# Autodesk Inventor assembly: Assembly
(part 2 of 3)
- C:\Users\Vincent Larson\Downloads\Universal_board_70x90mm_31x26\Universal_board_70x90mm_31x26-prt461.ipt
- C:\Users\Vincent Larson\Downloads\Universal_board_70x90mm_31x26\Universal_board_70x90mm_31x26-prt462.ipt
- C:\Users\Vincent Larson\Downloads\Universal_board_70x90mm_31x26\Universal_board_70x90mm_31x26-prt463.ipt
- C:\Users\Vincent Larson\Downloads\Universal_board_70x90mm_31x26\Universal_board_70x90mm_31x26-prt464.ipt
- C:\Users\Vincent Larson\Downloads\Universal_board_70x90mm_31x26\Universal_board_70x90mm_31x26-prt465.ipt
- C:\Users\Vincent Larson\Downloads\Universal_board_70x90mm_31x26\Universal_board_70x90mm_31x26-prt466.ipt
- C:\Users\Vincent Larson\Downloads\Universal_board_70x90mm_31x26\Universal_board_70x90mm_31x26-prt467.ipt
- C:\Users\Vincent Larson\Downloads\Universal_board_70x90mm_31x26\Universal_board_70x90mm_31x26-prt468.ipt
- C:\Users\Vincent Larson\Downloads\Universal_board_70x90mm_31x26\Universal_board_70x90mm_31x26-prt469.ipt
- C:\Users\Vincent Larson\Downloads\Universal_board_70x90mm_31x26\Universal_board_70x90mm_31x26-prt470.ipt
- C:\Users\Vincent Larson\Downloads\Universal_board_70x90mm_31x26\Universal_board_70x90mm_31x26-prt471.ipt
- C:\Users\Vincent Larson\Downloads\Universal_board_70x90mm_31x26\Universal_board_70x90mm_31x26-prt472.ipt
- C:\Users\Vincent Larson\Downloads\Universal_board_70x90mm_31x26\Universal_board_70x90mm_31x26-prt473.ipt
- C:\Users\Vincent Larson\Downloads\Universal_board_70x90mm_31x26\Universal_board_70x90mm_31x26-prt474.ipt
- C:\Users\Vincent Larson\Downloads\Universal_board_70x90mm_31x26\Universal_board_70x90mm_31x26-prt475.ipt
- C:\Users\Vincent Larson\Downloads\Universal_board_70x90mm_31x26\Universal_board_70x90mm_31x26-prt476.ipt
- C:\Users\Vincent Larson\Downloads\Universal_board_70x90mm_31x26\Universal_board_70x90mm_31x26-prt477.ipt
- C:\Users\Vincent Larson\Downloads\Universal_board_70x90mm_31x26\Universal_board_70x90mm_31x26-prt478.ipt
- C:\Users\Vincent Larson\Downloads\Universal_board_70x90mm_31x26\Universal_board_70x90mm_31x26-prt479.ipt
- C:\Users\Vincent Larson\Downloads\Universal_board_70x90mm_31x26\Universal_board_70x90mm_31x26-prt480.ipt
- C:\Users\Vincent Larson\Downloads\Universal_board_70x90mm_31x26\Universal_board_70x90mm_31x26-prt481.ipt
- C:\Users\Vincent Larson\Downloads\Universal_board_70x90mm_31x26\Universal_board_70x90mm_31x26-prt482.ipt
- C:\Users\Vincent Larson\Downloads\Universal_board_70x90mm_31x26\Universal_board_70x90mm_31x26-prt483.ipt
- C:\Users\Vincent Larson\Downloads\Universal_board_70x90mm_31x26\Universal_board_70x90mm_31x26-prt484.ipt
- C:\Users\Vincent Larson\Downloads\Universal_board_70x90mm_31x26\Universal_board_70x90mm_31x26-prt485.ipt
- C:\Users\Vincent Larson\Downloads\Universal_board_70x90mm_31x26\Universal_board_70x90mm_31x26-prt486.ipt
- C:\Users\Vincent Larson\Downloads\Universal_board_70x90mm_31x26\Universal_board_70x90mm_31x26-prt487.ipt
- C:\Users\Vincent Larson\Downloads\Universal_board_70x90mm_31x26\Universal_board_70x90mm_31x26-prt488.ipt
- C:\Users\Vincent Larson\Downloads\Universal_board_70x90mm_31x26\Universal_board_70x90mm_31x26-prt489.ipt
- C:\Users\Vincent Larson\Downloads\Universal_board_70x90mm_31x26\Universal_board_70x90mm_31x26-prt490.ipt
- C:\Users\Vincent Larson\Downloads\Universal_board_70x90mm_31x26\Universal_board_70x90mm_31x26-prt491.ipt
- C:\Users\Vincent Larson\Downloads\Universal_board_70x90mm_31x26\Universal_board_70x90mm_31x26-prt492.ipt
- C:\Users\Vincent Larson\Downloads\Universal_board_70x90mm_31x26\Universal_board_70x90mm_31x26-prt493.ipt
- C:\Users\Vincent Larson\Downloads\Universal_board_70x90mm_31x26\Universal_board_70x90mm_31x26-prt494.ipt
- C:\Users\Vincent Larson\Downloads\Universal_board_70x90mm_31x26\Universal_board_70x90mm_31x26-prt495.ipt
- C:\Users\Vincent Larson\Downloads\Universal_board_70x90mm_31x26\Universal_board_70x90mm_31x26-prt496.ipt
- C:\Users\Vincent Larson\Downloads\Universal_board_70x90mm_31x26\Universal_board_70x90mm_31x26-prt497.ipt
- C:\Users\Vincent Larson\Downloads\Universal_board_70x90mm_31x26\Universal_board_70x90mm_31x26-prt498.ipt
- C:\Users\Vincent Larson\Downloads\Universal_board_70x90mm_31x26\Universal_board_70x90mm_31x26-prt499.ipt
- C:\Users\Vincent Larson\Downloads\Universal_board_70x90mm_31x26\Universal_board_70x90mm_31x26-prt500.ipt
- C:\Users\Vincent Larson\Downloads\Universal_board_70x90mm_31x26\Universal_board_70x90mm_31x26-prt501.ipt
- C:\Users\Vincent Larson\Downloads\Universal_board_70x90mm_31x26\Universal_board_70x90mm_31x26-prt502.ipt
- C:\Users\Vincent Larson\Downloads\Universal_board_70x90mm_31x26\Universal_board_70x90mm_31x26-prt503.ipt
- C:\Users\Vincent Larson\Downloads\Universal_board_70x90mm_31x26\Universal_board_70x90mm_31x26-prt504.ipt
- C:\Users\Vincent Larson\Downloads\Universal_board_70x90mm_31x26\Universal_board_70x90mm_31x26-prt505.ipt
- C:\Users\Vincent Larson\Downloads\Universal_board_70x90mm_31x26\Universal_board_70x90mm_31x26-prt506.ipt
- C:\Users\Vincent Larson\Downloads\Universal_board_70x90mm_31x26\Universal_board_70x90mm_31x26-prt507.ipt
- C:\Users\Vincent Larson\Downloads\Universal_board_70x90mm_31x26\Universal_board_70x90mm_31x26-prt508.ipt
- C:\Users\Vincent Larson\Downloads\Universal_board_70x90mm_31x26\Universal_board_70x90mm_31x26-prt509.ipt
- C:\Users\Vincent Larson\Downloads\Universal_board_70x90mm_31x26\Universal_board_70x90mm_31x26-prt510.ipt
- C:\Users\Vincent Larson\Downloads\Universal_board_70x90mm_31x26\Universal_board_70x90mm_31x26-prt511.ipt
- C:\Users\Vincent Larson\Downloads\Universal_board_70x90mm_31x26\Universal_board_70x90mm_31x26-prt512.ipt
- C:\Users\Vincent Larson\Downloads\Universal_board_70x90mm_31x26\Universal_board_70x90mm_31x26-prt513.ipt
- C:\Users\Vincent Larson\Downloads\Universal_board_70x90mm_31x26\Universal_board_70x90mm_31x26-prt514.ipt
- C:\Users\Vincent Larson\Downloads\Universal_board_70x90mm_31x26\Universal_board_70x90mm_31x26-prt515.ipt
- C:\Users\Vincent Larson\Downloads\Universal_board_70x90mm_31x26\Universal_board_70x90mm_31x26-prt516.ipt
- C:\Users\Vincent Larson\Downloads\Universal_board_70x90mm_31x26\Universal_board_70x90mm_31x26-prt517.ipt
- C:\Users\Vincent Larson\Downloads\Universal_board_70x90mm_31x26\Universal_board_70x90mm_31x26-prt518.ipt
- C:\Users\Vincent Larson\Downloads\Universal_board_70x90mm_31x26\Universal_board_70x90mm_31x26-prt519.ipt
- C:\Users\Vincent Larson\Downloads\Universal_board_70x90mm_31x26\Universal_board_70x90mm_31x26-prt520.ipt
- C:\Users\Vincent Larson\Downloads\Universal_board_70x90mm_31x26\Universal_board_70x90mm_31x26-prt521.ipt
- C:\Users\Vincent Larson\Downloads\Universal_board_70x90mm_31x26\Universal_board_70x90mm_31x26-prt522.ipt
- C:\Users\Vincent Larson\Downloads\Universal_board_70x90mm_31x26\Universal_board_70x90mm_31x26-prt523.ipt
- C:\Users\Vincent Larson\Downloads\Universal_board_70x90mm_31x26\Universal_board_70x90mm_31x26-prt524.ipt
- C:\Users\Vincent Larson\Downloads\Universal_board_70x90mm_31x26\Universal_board_70x90mm_31x26-prt525.ipt
- C:\Users\Vincent Larson\Downloads\Universal_board_70x90mm_31x26\Universal_board_70x90mm_31x26-prt526.ipt
- C:\Users\Vincent Larson\Downloads\Universal_board_70x90mm_31x26\Universal_board_70x90mm_31x26-prt527.ipt
- C:\Users\Vincent Larson\Downloads\Universal_board_70x90mm_31x26\Universal_board_70x90mm_31x26-prt528.ipt
- C:\Users\Vincent Larson\Downloads\Universal_board_70x90mm_31x26\Universal_board_70x90mm_31x26-prt529.ipt
- C:\Users\Vincent Larson\Downloads\Universal_board_70x90mm_31x26\Universal_board_70x90mm_31x26-prt530.ipt
- C:\Users\Vincent Larson\Downloads\Universal_board_70x90mm_31x26\Universal_board_70x90mm_31x26-prt531.ipt
- C:\Users\Vincent Larson\Downloads\Universal_board_70x90mm_31x26\Universal_board_70x90mm_31x26-prt532.ipt
- C:\Users\Vincent Larson\Downloads\Universal_board_70x90mm_31x26\Universal_board_70x90mm_31x26-prt533.ipt
- C:\Users\Vincent Larson\Downloads\Universal_board_70x90mm_31x26\Universal_board_70x90mm_31x26-prt534.ipt
- C:\Users\Vincent Larson\Downloads\Universal_board_70x90mm_31x26\Universal_board_70x90mm_31x26-prt535.ipt
- C:\Users\Vincent Larson\Downloads\Universal_board_70x90mm_31x26\Universal_board_70x90mm_31x26-prt536.ipt
- C:\Users\Vincent Larson\Downloads\Universal_board_70x90mm_31x26\Universal_board_70x90mm_31x26-prt537.ipt
- C:\Users\Vincent Larson\Downloads\Universal_board_70x90mm_31x26\Universal_board_70x90mm_31x26-prt538.ipt
- C:\Users\Vincent Larson\Downloads\Universal_board_70x90mm_31x26\Universal_board_70x90mm_31x26-prt539.ipt
- C:\Users\Vincent Larson\Downloads\Universal_board_70x90mm_31x26\Universal_board_70x90mm_31x26-prt540.ipt
- C:\Users\Vincent Larson\Downloads\Universal_board_70x90mm_31x26\Universal_board_70x90mm_31x26-prt541.ipt
- C:\Users\Vincent Larson\Downloads\Universal_board_70x90mm_31x26\Universal_board_70x90mm_31x26-prt542.ipt
- C:\Users\Vincent Larson\Downloads\Universal_board_70x90mm_31x26\Universal_board_70x90mm_31x26-prt543.ipt
- C:\Users\Vincent Larson\Downloads\Universal_board_70x90mm_31x26\Universal_board_70x90mm_31x26-prt544.ipt
- C:\Users\Vincent Larson\Downloads\Universal_board_70x90mm_31x26\Universal_board_70x90mm_31x26-prt545.ipt
- C:\Users\Vincent Larson\Downloads\Universal_board_70x90mm_31x26\Universal_board_70x90mm_31x26-prt546.ipt
- C:\Users\Vincent Larson\Downloads\Universal_board_70x90mm_31x26\Universal_board_70x90mm_31x26-prt547.ipt
- C:\Users\Vincent Larson\Downloads\Universal_board_70x90mm_31x26\Universal_board_70x90mm_31x26-prt548.ipt
- C:\Users\Vincent Larson\Downloads\Universal_board_70x90mm_31x26\Universal_board_70x90mm_31x26-prt549.ipt
- C:\Users\Vincent Larson\Downloads\Universal_board_70x90mm_31x26\Universal_board_70x90mm_31x26-prt550.ipt
- C:\Users\Vincent Larson\Downloads\Universal_board_70x90mm_31x26\Universal_board_70x90mm_31x26-prt551.ipt
- C:\Users\Vincent Larson\Downloads\Universal_board_70x90mm_31x26\Universal_board_70x90mm_31x26-prt552.ipt
- C:\Users\Vincent Larson\Downloads\Universal_board_70x90mm_31x26\Universal_board_70x90mm_31x26-prt553.ipt
- C:\Users\Vincent Larson\Downloads\Universal_board_70x90mm_31x26\Universal_board_70x90mm_31x26-prt554.ipt
- C:\Users\Vincent Larson\Downloads\Universal_board_70x90mm_31x26\Universal_board_70x90mm_31x26-prt555.ipt
- C:\Users\Vincent Larson\Downloads\Universal_board_70x90mm_31x26\Universal_board_70x90mm_31x26-prt556.ipt
- C:\Users\Vincent Larson\Downloads\Universal_board_70x90mm_31x26\Universal_board_70x90mm_31x26-prt557.ipt
- C:\Users\Vincent Larson\Downloads\Universal_board_70x90mm_31x26\Universal_board_70x90mm_31x26-prt558.ipt
- C:\Users\Vincent Larson\Downloads\Universal_board_70x90mm_31x26\Universal_board_70x90mm_31x26-prt559.ipt
- C:\Users\Vincent Larson\Downloads\Universal_board_70x90mm_31x26\Universal_board_70x90mm_31x26-prt560.ipt
- C:\Users\Vincent Larson\Downloads\Universal_board_70x90mm_31x26\Universal_board_70x90mm_31x26-prt561.ipt
- C:\Users\Vincent Larson\Downloads\Universal_board_70x90mm_31x26\Universal_board_70x90mm_31x26-prt562.ipt
- C:\Users\Vincent Larson\Downloads\Universal_board_70x90mm_31x26\Universal_board_70x90mm_31x26-prt563.ipt
- C:\Users\Vincent Larson\Downloads\Universal_board_70x90mm_31x26\Universal_board_70x90mm_31x26-prt564.ipt
- C:\Users\Vincent Larson\Downloads\Universal_board_70x90mm_31x26\Universal_board_70x90mm_31x26-prt565.ipt
- C:\Users\Vincent Larson\Downloads\Universal_board_70x90mm_31x26\Universal_board_70x90mm_31x26-prt566.ipt
- C:\Users\Vincent Larson\Downloads\Universal_board_70x90mm_31x26\Universal_board_70x90mm_31x26-prt567.ipt
- C:\Users\Vincent Larson\Downloads\Universal_board_70x90mm_31x26\Universal_board_70x90mm_31x26-prt568.ipt
- C:\Users\Vincent Larson\Downloads\Universal_board_70x90mm_31x26\Universal_board_70x90mm_31x26-prt569.ipt
- C:\Users\Vincent Larson\Downloads\Universal_board_70x90mm_31x26\Universal_board_70x90mm_31x26-prt570.ipt
- C:\Users\Vincent Larson\Downloads\Universal_board_70x90mm_31x26\Universal_board_70x90mm_31x26-prt571.ipt
- C:\Users\Vincent Larson\Downloads\Universal_board_70x90mm_31x26\Universal_board_70x90mm_31x26-prt572.ipt
- C:\Users\Vincent Larson\Downloads\Universal_board_70x90mm_31x26\Universal_board_70x90mm_31x26-prt573.ipt
- C:\Users\Vincent Larson\Downloads\Universal_board_70x90mm_31x26\Universal_board_70x90mm_31x26-prt574.ipt
- C:\Users\Vincent Larson\Downloads\Universal_board_70x90mm_31x26\Universal_board_70x90mm_31x26-prt575.ipt
- C:\Users\Vincent Larson\Downloads\Universal_board_70x90mm_31x26\Universal_board_70x90mm_31x26-prt576.ipt
- C:\Users\Vincent Larson\Downloads\Universal_board_70x90mm_31x26\Universal_board_70x90mm_31x26-prt577.ipt
- C:\Users\Vincent Larson\Downloads\Universal_board_70x90mm_31x26\Universal_board_70x90mm_31x26-prt578.ipt
- C:\Users\Vincent Larson\Downloads\Universal_board_70x90mm_31x26\Universal_board_70x90mm_31x26-prt579.ipt
- C:\Users\Vincent Larson\Downloads\Universal_board_70x90mm_31x26\Universal_board_70x90mm_31x26-prt580.ipt
- C:\Users\Vincent Larson\Downloads\Universal_board_70x90mm_31x26\Universal_board_70x90mm_31x26-prt581.ipt
- C:\Users\Vincent Larson\Downloads\Universal_board_70x90mm_31x26\Universal_board_70x90mm_31x26-prt582.ipt
- C:\Users\Vincent Larson\Downloads\Universal_board_70x90mm_31x26\Universal_board_70x90mm_31x26-prt583.ipt
- C:\Users\Vincent Larson\Downloads\Universal_board_70x90mm_31x26\Universal_board_70x90mm_31x26-prt584.ipt
- C:\Users\Vincent Larson\Downloads\Universal_board_70x90mm_31x26\Universal_board_70x90mm_31x26-prt585.ipt
- C:\Users\Vincent Larson\Downloads\Universal_board_70x90mm_31x26\Universal_board_70x90mm_31x26-prt586.ipt
- C:\Users\Vincent Larson\Downloads\Universal_board_70x90mm_31x26\Universal_board_70x90mm_31x26-prt587.ipt
- C:\Users\Vincent Larson\Downloads\Universal_board_70x90mm_31x26\Universal_board_70x90mm_31x26-prt588.ipt
- C:\Users\Vincent Larson\Downloads\Universal_board_70x90mm_31x26\Universal_board_70x90mm_31x26-prt589.ipt
- C:\Users\Vincent Larson\Downloads\Universal_board_70x90mm_31x26\Universal_board_70x90mm_31x26-prt590.ipt
- C:\Users\Vincent Larson\Downloads\Universal_board_70x90mm_31x26\Universal_board_70x90mm_31x26-prt591.ipt
- C:\Users\Vincent Larson\Downloads\Universal_board_70x90mm_31x26\Universal_board_70x90mm_31x26-prt592.ipt
- C:\Users\Vincent Larson\Downloads\Universal_board_70x90mm_31x26\Universal_board_70x90mm_31x26-prt593.ipt
- C:\Users\Vincent Larson\Downloads\Universal_board_70x90mm_31x26\Universal_board_70x90mm_31x26-prt594.ipt
- C:\Users\Vincent Larson\Downloads\Universal_board_70x90mm_31x26\Universal_board_70x90mm_31x26-prt595.ipt
- C:\Users\Vincent Larson\Downloads\Universal_board_70x90mm_31x26\Universal_board_70x90mm_31x26-prt596.ipt
- C:\Users\Vincent Larson\Downloads\Universal_board_70x90mm_31x26\Universal_board_70x90mm_31x26-prt597.ipt
- C:\Users\Vincent Larson\Downloads\Universal_board_70x90mm_31x26\Universal_board_70x90mm_31x26-prt598.ipt
- C:\Users\Vincent Larson\Downloads\Universal_board_70x90mm_31x26\Universal_board_70x90mm_31x26-prt599.ipt
- C:\Users\Vincent Larson\Downloads\Universal_board_70x90mm_31x26\Universal_board_70x90mm_31x26-prt600.ipt
- C:\Users\Vincent Larson\Downloads\Universal_board_70x90mm_31x26\Universal_board_70x90mm_31x26-prt601.ipt
- C:\Users\Vincent Larson\Downloads\Universal_board_70x90mm_31x26\Universal_board_70x90mm_31x26-prt602.ipt
- C:\Users\Vincent Larson\Downloads\Universal_board_70x90mm_31x26\Universal_board_70x90mm_31x26-prt603.ipt
- C:\Users\Vincent Larson\Downloads\Universal_board_70x90mm_31x26\Universal_board_70x90mm_31x26-prt604.ipt
- C:\Users\Vincent Larson\Downloads\Universal_board_70x90mm_31x26\Universal_board_70x90mm_31x26-prt605.ipt
- C:\Users\Vincent Larson\Downloads\Universal_board_70x90mm_31x26\Universal_board_70x90mm_31x26-prt606.ipt
- C:\Users\Vincent Larson\Downloads\Universal_board_70x90mm_31x26\Universal_board_70x90mm_31x26-prt607.ipt
- C:\Users\Vincent Larson\Downloads\Universal_board_70x90mm_31x26\Universal_board_70x90mm_31x26-prt608.ipt
- C:\Users\Vincent Larson\Downloads\Universal_board_70x90mm_31x26\Universal_board_70x90mm_31x26-prt609.ipt
- C:\Users\Vincent Larson\Downloads\Universal_board_70x90mm_31x26\Universal_board_70x90mm_31x26-prt610.ipt
- C:\Users\Vincent Larson\Downloads\Universal_board_70x90mm_31x26\Universal_board_70x90mm_31x26-prt611.ipt
- C:\Users\Vincent Larson\Downloads\Universal_board_70x90mm_31x26\Universal_board_70x90mm_31x26-prt612.ipt
- C:\Users\Vincent Larson\Downloads\Universal_board_70x90mm_31x26\Universal_board_70x90mm_31x26-prt613.ipt
- C:\Users\Vincent Larson\Downloads\Universal_board_70x90mm_31x26\Universal_board_70x90mm_31x26-prt614.ipt
- C:\Users\Vincent Larson\Downloads\Universal_board_70x90mm_31x26\Universal_board_70x90mm_31x26-prt615.ipt
- C:\Users\Vincent Larson\Downloads\Universal_board_70x90mm_31x26\Universal_board_70x90mm_31x26-prt616.ipt
- C:\Users\Vincent Larson\Downloads\Universal_board_70x90mm_31x26\Universal_board_70x90mm_31x26-prt617.ipt
- C:\Users\Vincent Larson\Downloads\Universal_board_70x90mm_31x26\Universal_board_70x90mm_31x26-prt618.ipt
- C:\Users\Vincent Larson\Downloads\Universal_board_70x90mm_31x26\Universal_board_70x90mm_31x26-prt619.ipt
- C:\Users\Vincent Larson\Downloads\Universal_board_70x90mm_31x26\Universal_board_70x90mm_31x26-prt620.ipt
- C:\Users\Vincent Larson\Downloads\Universal_board_70x90mm_31x26\Universal_board_70x90mm_31x26-prt621.ipt
- C:\Users\Vincent Larson\Downloads\Universal_board_70x90mm_31x26\Universal_board_70x90mm_31x26-prt622.ipt
- C:\Users\Vincent Larson\Downloads\Universal_board_70x90mm_31x26\Universal_board_70x90mm_31x26-prt623.ipt
- C:\Users\Vincent Larson\Downloads\Universal_board_70x90mm_31x26\Universal_board_70x90mm_31x26-prt624.ipt
- C:\Users\Vincent Larson\Downloads\Universal_board_70x90mm_31x26\Universal_board_70x90mm_31x26-prt625.ipt
- C:\Users\Vincent Larson\Downloads\Universal_board_70x90mm_31x26\Universal_board_70x90mm_31x26-prt626.ipt
- C:\Users\Vincent Larson\Downloads\Universal_board_70x90mm_31x26\Universal_board_70x90mm_31x26-prt627.ipt
- C:\Users\Vincent Larson\Downloads\Universal_board_70x90mm_31x26\Universal_board_70x90mm_31x26-prt628.ipt
- C:\Users\Vincent Larson\Downloads\Universal_board_70x90mm_31x26\Universal_board_70x90mm_31x26-prt629.ipt
- C:\Users\Vincent Larson\Downloads\Universal_board_70x90mm_31x26\Universal_board_70x90mm_31x26-prt630.ipt
- C:\Users\Vincent Larson\Downloads\Universal_board_70x90mm_31x26\Universal_board_70x90mm_31x26-prt631.ipt
- C:\Users\Vincent Larson\Downloads\Universal_board_70x90mm_31x26\Universal_board_70x90mm_31x26-prt632.ipt
- C:\Users\Vincent Larson\Downloads\Universal_board_70x90mm_31x26\Universal_board_70x90mm_31x26-prt633.ipt
- C:\Users\Vincent Larson\Downloads\Universal_board_70x90mm_31x26\Universal_board_70x90mm_31x26-prt634.ipt
- C:\Users\Vincent Larson\Downloads\Universal_board_70x90mm_31x26\Universal_board_70x90mm_31x26-prt635.ipt
- C:\Users\Vincent Larson\Downloads\Universal_board_70x90mm_31x26\Universal_board_70x90mm_31x26-prt636.ipt
- C:\Users\Vincent Larson\Downloads\Universal_board_70x90mm_31x26\Universal_board_70x90mm_31x26-prt637.ipt
- C:\Users\Vincent Larson\Downloads\Universal_board_70x90mm_31x26\Universal_board_70x90mm_31x26-prt638.ipt
- C:\Users\Vincent Larson\Downloads\Universal_board_70x90mm_31x26\Universal_board_70x90mm_31x26-prt639.ipt
- C:\Users\Vincent Larson\Downloads\Universal_board_70x90mm_31x26\Universal_board_70x90mm_31x26-prt640.ipt
- C:\Users\Vincent Larson\Downloads\Universal_board_70x90mm_31x26\Universal_board_70x90mm_31x26-prt641.ipt
- C:\Users\Vincent Larson\Downloads\Universal_board_70x90mm_31x26\Universal_board_70x90mm_31x26-prt642.ipt
- C:\Users\Vincent Larson\Downloads\Universal_board_70x90mm_31x26\Universal_board_70x90mm_31x26-prt643.ipt
- C:\Users\Vincent Larson\Downloads\Universal_board_70x90mm_31x26\Universal_board_70x90mm_31x26-prt644.ipt
- C:\Users\Vincent Larson\Downloads\Universal_board_70x90mm_31x26\Universal_board_70x90mm_31x26-prt645.ipt
- C:\Users\Vincent Larson\Downloads\Universal_board_70x90mm_31x26\Universal_board_70x90mm_31x26-prt646.ipt
- C:\Users\Vincent Larson\Downloads\Universal_board_70x90mm_31x26\Universal_board_70x90mm_31x26-prt647.ipt
- C:\Users\Vincent Larson\Downloads\Universal_board_70x90mm_31x26\Universal_board_70x90mm_31x26-prt648.ipt
- C:\Users\Vincent Larson\Downloads\Universal_board_70x90mm_31x26\Universal_board_70x90mm_31x26-prt649.ipt
- C:\Users\Vincent Larson\Downloads\Universal_board_70x90mm_31x26\Universal_board_70x90mm_31x26-prt650.ipt
- C:\Users\Vincent Larson\Downloads\Universal_board_70x90mm_31x26\Universal_board_70x90mm_31x26-prt651.ipt
- C:\Users\Vincent Larson\Downloads\Universal_board_70x90mm_31x26\Universal_board_70x90mm_31x26-prt652.ipt
- C:\Users\Vincent Larson\Downloads\Universal_board_70x90mm_31x26\Universal_board_70x90mm_31x26-prt653.ipt
- C:\Users\Vincent Larson\Downloads\Universal_board_70x90mm_31x26\Universal_board_70x90mm_31x26-prt654.ipt
- C:\Users\Vincent Larson\Downloads\Universal_board_70x90mm_31x26\Universal_board_70x90mm_31x26-prt655.ipt
- C:\Users\Vincent Larson\Downloads\Universal_board_70x90mm_31x26\Universal_board_70x90mm_31x26-prt656.ipt
- C:\Users\Vincent Larson\Downloads\Universal_board_70x90mm_31x26\Universal_board_70x90mm_31x26-prt657.ipt
- C:\Users\Vincent Larson\Downloads\Universal_board_70x90mm_31x26\Universal_board_70x90mm_31x26-prt658.ipt
- C:\Users\Vincent Larson\Downloads\Universal_board_70x90mm_31x26\Universal_board_70x90mm_31x26-prt659.ipt
- C:\Users\Vincent Larson\Downloads\Universal_board_70x90mm_31x26\Universal_board_70x90mm_31x26-prt660.ipt
- C:\Users\Vincent Larson\Downloads\Universal_board_70x90mm_31x26\Universal_board_70x90mm_31x26-prt661.ipt
- C:\Users\Vincent Larson\Downloads\Universal_board_70x90mm_31x26\Universal_board_70x90mm_31x26-prt662.ipt
- C:\Users\Vincent Larson\Downloads\Universal_board_70x90mm_31x26\Universal_board_70x90mm_31x26-prt663.ipt
- C:\Users\Vincent Larson\Downloads\Universal_board_70x90mm_31x26\Universal_board_70x90mm_31x26-prt664.ipt
- C:\Users\Vincent Larson\Downloads\Universal_board_70x90mm_31x26\Universal_board_70x90mm_31x26-prt665.ipt
- C:\Users\Vincent Larson\Downloads\Universal_board_70x90mm_31x26\Universal_board_70x90mm_31x26-prt666.ipt
- C:\Users\Vincent Larson\Downloads\Universal_board_70x90mm_31x26\Universal_board_70x90mm_31x26-prt667.ipt
- C:\Users\Vincent Larson\Downloads\Universal_board_70x90mm_31x26\Universal_board_70x90mm_31x26-prt668.ipt
- C:\Users\Vincent Larson\Downloads\Universal_board_70x90mm_31x26\Universal_board_70x90mm_31x26-prt669.ipt
- C:\Users\Vincent Larson\Downloads\Universal_board_70x90mm_31x26\Universal_board_70x90mm_31x26-prt670.ipt
- C:\Users\Vincent Larson\Downloads\Universal_board_70x90mm_31x26\Universal_board_70x90mm_31x26-prt671.ipt
- C:\Users\Vincent Larson\Downloads\Universal_board_70x90mm_31x26\Universal_board_70x90mm_31x26-prt672.ipt
- C:\Users\Vincent Larson\Downloads\Universal_board_70x90mm_31x26\Universal_board_70x90mm_31x26-prt673.ipt
- C:\Users\Vincent Larson\Downloads\Universal_board_70x90mm_31x26\Universal_board_70x90mm_31x26-prt674.ipt
- C:\Users\Vincent Larson\Downloads\Universal_board_70x90mm_31x26\Universal_board_70x90mm_31x26-prt675.ipt
- C:\Users\Vincent Larson\Downloads\Universal_board_70x90mm_31x26\Universal_board_70x90mm_31x26-prt676.ipt
- C:\Users\Vincent Larson\Downloads\Universal_board_70x90mm_31x26\Universal_board_70x90mm_31x26-prt677.ipt
- C:\Users\Vincent Larson\Downloads\Universal_board_70x90mm_31x26\Universal_board_70x90mm_31x26-prt678.ipt
- C:\Users\Vincent Larson\Downloads\Universal_board_70x90mm_31x26\Universal_board_70x90mm_31x26-prt679.ipt
- C:\Users\Vincent Larson\Downloads\Universal_board_70x90mm_31x26\Universal_board_70x90mm_31x26-prt680.ipt
- C:\Users\Vincent Larson\Downloads\Universal_board_70x90mm_31x26\Universal_board_70x90mm_31x26-prt681.ipt
- C:\Users\Vincent Larson\Downloads\Universal_board_70x90mm_31x26\Universal_board_70x90mm_31x26-prt682.ipt
- C:\Users\Vincent Larson\Downloads\Universal_board_70x90mm_31x26\Universal_board_70x90mm_31x26-prt683.ipt
- C:\Users\Vincent Larson\Downloads\Universal_board_70x90mm_31x26\Universal_board_70x90mm_31x26-prt684.ipt
- C:\Users\Vincent Larson\Downloads\Universal_board_70x90mm_31x26\Universal_board_70x90mm_31x26-prt685.ipt
- C:\Users\Vincent Larson\Downloads\Universal_board_70x90mm_31x26\Universal_board_70x90mm_31x26-prt686.ipt
- C:\Users\Vincent Larson\Downloads\Universal_board_70x90mm_31x26\Universal_board_70x90mm_31x26-prt687.ipt
- C:\Users\Vincent Larson\Downloads\Universal_board_70x90mm_31x26\Universal_board_70x90mm_31x26-prt688.ipt
- C:\Users\Vincent Larson\Downloads\Universal_board_70x90mm_31x26\Universal_board_70x90mm_31x26-prt689.ipt
- C:\Users\Vincent Larson\Downloads\Universal_board_70x90mm_31x26\Universal_board_70x90mm_31x26-prt690.ipt
- C:\Users\Vincent Larson\Downloads\Universal_board_70x90mm_31x26\Universal_board_70x90mm_31x26-prt691.ipt
- C:\Users\Vincent Larson\Downloads\Universal_board_70x90mm_31x26\Universal_board_70x90mm_31x26-prt692.ipt
- C:\Users\Vincent Larson\Downloads\Universal_board_70x90mm_31x26\Universal_board_70x90mm_31x26-prt693.ipt
- C:\Users\Vincent Larson\Downloads\Universal_board_70x90mm_31x26\Universal_board_70x90mm_31x26-prt694.ipt
- C:\Users\Vincent Larson\Downloads\Universal_board_70x90mm_31x26\Universal_board_70x90mm_31x26-prt695.ipt
- C:\Users\Vincent Larson\Downloads\Universal_board_70x90mm_31x26\Universal_board_70x90mm_31x26-prt696.ipt
- C:\Users\Vincent Larson\Downloads\Universal_board_70x90mm_31x26\Universal_board_70x90mm_31x26-prt697.ipt
- C:\Users\Vincent Larson\Downloads\Universal_board_70x90mm_31x26\Universal_board_70x90mm_31x26-prt698.ipt
- C:\Users\Vincent Larson\Downloads\Universal_board_70x90mm_31x26\Universal_board_70x90mm_31x26-prt699.ipt
- C:\Users\Vincent Larson\Downloads\Universal_board_70x90mm_31x26\Universal_board_70x90mm_31x26-prt700.ipt
- C:\Users\Vincent Larson\Downloads\Universal_board_70x90mm_31x26\Universal_board_70x90mm_31x26-prt701.ipt
- C:\Users\Vincent Larson\Downloads\Universal_board_70x90mm_31x26\Universal_board_70x90mm_31x26-prt702.ipt
- C:\Users\Vincent Larson\Downloads\Universal_board_70x90mm_31x26\Universal_board_70x90mm_31x26-prt703.ipt
- C:\Users\Vincent Larson\Downloads\Universal_board_70x90mm_31x26\Universal_board_70x90mm_31x26-prt704.ipt
- C:\Users\Vincent Larson\Downloads\Universal_board_70x90mm_31x26\Universal_board_70x90mm_31x26-prt705.ipt
- C:\Users\Vincent Larson\Downloads\Universal_board_70x90mm_31x26\Universal_board_70x90mm_31x26-prt706.ipt
- C:\Users\Vincent Larson\Downloads\Universal_board_70x90mm_31x26\Universal_board_70x90mm_31x26-prt707.ipt
- C:\Users\Vincent Larson\Downloads\Universal_board_70x90mm_31x26\Universal_board_70x90mm_31x26-prt708.ipt
- C:\Users\Vincent Larson\Downloads\Universal_board_70x90mm_31x26\Universal_board_70x90mm_31x26-prt709.ipt
- C:\Users\Vincent Larson\Downloads\Universal_board_70x90mm_31x26\Universal_board_70x90mm_31x26-prt710.ipt
- C:\Users\Vincent Larson\Downloads\Universal_board_70x90mm_31x26\Universal_board_70x90mm_31x26-prt711.ipt
- C:\Users\Vincent Larson\Downloads\Universal_board_70x90mm_31x26\Universal_board_70x90mm_31x26-prt712.ipt
- C:\Users\Vincent Larson\Downloads\Universal_board_70x90mm_31x26\Universal_board_70x90mm_31x26-prt713.ipt
- C:\Users\Vincent Larson\Downloads\Universal_board_70x90mm_31x26\Universal_board_70x90mm_31x26-prt714.ipt
- C:\Users\Vincent Larson\Downloads\Universal_board_70x90mm_31x26\Universal_board_70x90mm_31x26-prt715.ipt
- C:\Users\Vincent Larson\Downloads\Universal_board_70x90mm_31x26\Universal_board_70x90mm_31x26-prt716.ipt
- C:\Users\Vincent Larson\Downloads\Universal_board_70x90mm_31x26\Universal_board_70x90mm_31x26-prt717.ipt
- C:\Users\Vincent Larson\Downloads\Universal_board_70x90mm_31x26\Universal_board_70x90mm_31x26-prt718.ipt
- C:\Users\Vincent Larson\Downloads\Universal_board_70x90mm_31x26\Universal_board_70x90mm_31x26-prt719.ipt
- C:\Users\Vincent Larson\Downloads\Universal_board_70x90mm_31x26\Universal_board_70x90mm_31x26-prt720.ipt
- C:\Users\Vincent Larson\Downloads\Universal_board_70x90mm_31x26\Universal_board_70x90mm_31x26-prt721.ipt
- C:\Users\Vincent Larson\Downloads\Universal_board_70x90mm_31x26\Universal_board_70x90mm_31x26-prt722.ipt
- C:\Users\Vincent Larson\Downloads\Universal_board_70x90mm_31x26\Universal_board_70x90mm_31x26-prt723.ipt
- C:\Users\Vincent Larson\Downloads\Universal_board_70x90mm_31x26\Universal_board_70x90mm_31x26-prt724.ipt
- C:\Users\Vincent Larson\Downloads\Universal_board_70x90mm_31x26\Universal_board_70x90mm_31x26-prt725.ipt
- C:\Users\Vincent Larson\Downloads\Universal_board_70x90mm_31x26\Universal_board_70x90mm_31x26-prt726.ipt
- C:\Users\Vincent Larson\Downloads\Universal_board_70x90mm_31x26\Universal_board_70x90mm_31x26-prt727.ipt
- C:\Users\Vincent Larson\Downloads\Universal_board_70x90mm_31x26\Universal_board_70x90mm_31x26-prt728.ipt
- C:\Users\Vincent Larson\Downloads\Universal_board_70x90mm_31x26\Universal_board_70x90mm_31x26-prt729.ipt
- C:\Users\Vincent Larson\Downloads\Universal_board_70x90mm_31x26\Universal_board_70x90mm_31x26-prt730.ipt
- C:\Users\Vincent Larson\Downloads\Universal_board_70x90mm_31x26\Universal_board_70x90mm_31x26-prt731.ipt
- C:\Users\Vincent Larson\Downloads\Universal_board_70x90mm_31x26\Universal_board_70x90mm_31x26-prt732.ipt
- C:\Users\Vincent Larson\Downloads\Universal_board_70x90mm_31x26\Universal_board_70x90mm_31x26-prt733.ipt
- C:\Users\Vincent Larson\Downloads\Universal_board_70x90mm_31x26\Universal_board_70x90mm_31x26-prt734.ipt
- C:\Users\Vincent Larson\Downloads\Universal_board_70x90mm_31x26\Universal_board_70x90mm_31x26-prt735.ipt
- C:\Users\Vincent Larson\Downloads\Universal_board_70x90mm_31x26\Universal_board_70x90mm_31x26-prt736.ipt
- C:\Users\Vincent Larson\Downloads\Universal_board_70x90mm_31x26\Universal_board_70x90mm_31x26-prt737.ipt
- C:\Users\Vincent Larson\Downloads\Universal_board_70x90mm_31x26\Universal_board_70x90mm_31x26-prt738.ipt
- C:\Users\Vincent Larson\Downloads\Universal_board_70x90mm_31x26\Universal_board_70x90mm_31x26-prt739.ipt
- C:\Users\Vincent Larson\Downloads\Universal_board_70x90mm_31x26\Universal_board_70x90mm_31x26-prt740.ipt
- C:\Users\Vincent Larson\Downloads\Universal_board_70x90mm_31x26\Universal_board_70x90mm_31x26-prt741.ipt
- C:\Users\Vincent Larson\Downloads\Universal_board_70x90mm_31x26\Universal_board_70x90mm_31x26-prt742.ipt
- C:\Users\Vincent Larson\Downloads\Universal_board_70x90mm_31x26\Universal_board_70x90mm_31x26-prt743.ipt
- C:\Users\Vincent Larson\Downloads\Universal_board_70x90mm_31x26\Universal_board_70x90mm_31x26-prt744.ipt
- C:\Users\Vincent Larson\Downloads\Universal_board_70x90mm_31x26\Universal_board_70x90mm_31x26-prt745.ipt
- C:\Users\Vincent Larson\Downloads\Universal_board_70x90mm_31x26\Universal_board_70x90mm_31x26-prt746.ipt
- C:\Users\Vincent Larson\Downloads\Universal_board_70x90mm_31x26\Universal_board_70x90mm_31x26-prt747.ipt
- C:\Users\Vincent Larson\Downloads\Universal_board_70x90mm_31x26\Universal_board_70x90mm_31x26-prt748.ipt
- C:\Users\Vincent Larson\Downloads\Universal_board_70x90mm_31x26\Universal_board_70x90mm_31x26-prt749.ipt
- C:\Users\Vincent Larson\Downloads\Universal_board_70x90mm_31x26\Universal_board_70x90mm_31x26-prt750.ipt
- C:\Users\Vincent Larson\Downloads\Universal_board_70x90mm_31x26\Universal_board_70x90mm_31x26-prt751.ipt
- C:\Users\Vincent Larson\Downloads\Universal_board_70x90mm_31x26\Universal_board_70x90mm_31x26-prt752.ipt
- C:\Users\Vincent Larson\Downloads\Universal_board_70x90mm_31x26\Universal_board_70x90mm_31x26-prt753.ipt
- C:\Users\Vincent Larson\Downloads\Universal_board_70x90mm_31x26\Universal_board_70x90mm_31x26-prt754.ipt
- C:\Users\Vincent Larson\Downloads\Universal_board_70x90mm_31x26\Universal_board_70x90mm_31x26-prt755.ipt
- C:\Users\Vincent Larson\Downloads\Universal_board_70x90mm_31x26\Universal_board_70x90mm_31x26-prt756.ipt
- C:\Users\Vincent Larson\Downloads\Universal_board_70x90mm_31x26\Universal_board_70x90mm_31x26-prt757.ipt
- C:\Users\Vincent Larson\Downloads\Universal_board_70x90mm_31x26\Universal_board_70x90mm_31x26-prt758.ipt
- C:\Users\Vincent Larson\Downloads\Universal_board_70x90mm_31x26\Universal_board_70x90mm_31x26-prt759.ipt
- C:\Users\Vincent Larson\Downloads\Universal_board_70x90mm_31x26\Universal_board_70x90mm_31x26-prt760.ipt
- C:\Users\Vincent Larson\Downloads\Universal_board_70x90mm_31x26\Universal_board_70x90mm_31x26-prt761.ipt
- C:\Users\Vincent Larson\Downloads\Universal_board_70x90mm_31x26\Universal_board_70x90mm_31x26-prt762.ipt
- C:\Users\Vincent Larson\Downloads\Universal_board_70x90mm_31x26\Universal_board_70x90mm_31x26-prt763.ipt
- C:\Users\Vincent Larson\Downloads\Universal_board_70x90mm_31x26\Universal_board_70x90mm_31x26-prt764.ipt
- C:\Users\Vincent Larson\Downloads\Universal_board_70x90mm_31x26\Universal_board_70x90mm_31x26-prt765.ipt
- C:\Users\Vincent Larson\Downloads\Universal_board_70x90mm_31x26\Universal_board_70x90mm_31x26-prt766.ipt
- C:\Users\Vincent Larson\Downloads\Universal_board_70x90mm_31x26\Universal_board_70x90mm_31x26-prt767.ipt
- C:\Users\Vincent Larson\Downloads\Universal_board_70x90mm_31x26\Universal_board_70x90mm_31x26-prt768.ipt
- C:\Users\Vincent Larson\Downloads\Universal_board_70x90mm_31x26\Universal_board_70x90mm_31x26-prt769.ipt
- C:\Users\Vincent Larson\Downloads\Universal_board_70x90mm_31x26\Universal_board_70x90mm_31x26-prt770.ipt
- C:\Users\Vincent Larson\Downloads\Universal_board_70x90mm_31x26\Universal_board_70x90mm_31x26-prt771.ipt
- C:\Users\Vincent Larson\Downloads\Universal_board_70x90mm_31x26\Universal_board_70x90mm_31x26-prt772.ipt
- C:\Users\Vincent Larson\Downloads\Universal_board_70x90mm_31x26\Universal_board_70x90mm_31x26-prt773.ipt
- C:\Users\Vincent Larson\Downloads\Universal_board_70x90mm_31x26\Universal_board_70x90mm_31x26-prt774.ipt
- C:\Users\Vincent Larson\Downloads\Universal_board_70x90mm_31x26\Universal_board_70x90mm_31x26-prt775.ipt
- C:\Users\Vincent Larson\Downloads\Universal_board_70x90mm_31x26\Universal_board_70x90mm_31x26-prt776.ipt
- C:\Users\Vincent Larson\Downloads\Universal_board_70x90mm_31x26\Universal_board_70x90mm_31x26-prt777.ipt
- C:\Users\Vincent Larson\Downloads\Universal_board_70x90mm_31x26\Universal_board_70x90mm_31x26-prt778.ipt
- C:\Users\Vincent Larson\Downloads\Universal_board_70x90mm_31x26\Universal_board_70x90mm_31x26-prt779.ipt
- C:\Users\Vincent Larson\Downloads\Universal_board_70x90mm_31x26\Universal_board_70x90mm_31x26-prt780.ipt
- C:\Users\Vincent Larson\Downloads\Universal_board_70x90mm_31x26\Universal_board_70x90mm_31x26-prt781.ipt
- C:\Users\Vincent Larson\Downloads\Universal_board_70x90mm_31x26\Universal_board_70x90mm_31x26-prt782.ipt
- C:\Users\Vincent Larson\Downloads\Universal_board_70x90mm_31x26\Universal_board_70x90mm_31x26-prt783.ipt
- C:\Users\Vincent Larson\Downloads\Universal_board_70x90mm_31x26\Universal_board_70x90mm_31x26-prt784.ipt
- C:\Users\Vincent Larson\Downloads\Universal_board_70x90mm_31x26\Universal_board_70x90mm_31x26-prt785.ipt
- C:\Users\Vincent Larson\Downloads\Universal_board_70x90mm_31x26\Universal_board_70x90mm_31x26-prt786.ipt
- C:\Users\Vincent Larson\Downloads\Universal_board_70x90mm_31x26\Universal_board_70x90mm_31x26-prt787.ipt
- C:\Users\Vincent Larson\Downloads\Universal_board_70x90mm_31x26\Universal_board_70x90mm_31x26-prt788.ipt
- C:\Users\Vincent Larson\Downloads\Universal_board_70x90mm_31x26\Universal_board_70x90mm_31x26-prt789.ipt
- C:\Users\Vincent Larson\Downloads\Universal_board_70x90mm_31x26\Universal_board_70x90mm_31x26-prt790.ipt
- C:\Users\Vincent Larson\Downloads\Universal_board_70x90mm_31x26\Universal_board_70x90mm_31x26-prt791.ipt
- C:\Users\Vincent Larson\Downloads\Universal_board_70x90mm_31x26\Universal_board_70x90mm_31x26-prt792.ipt
- C:\Users\Vincent Larson\Downloads\Universal_board_70x90mm_31x26\Universal_board_70x90mm_31x26-prt793.ipt
- C:\Users\Vincent Larson\Downloads\Universal_board_70x90mm_31x26\Universal_board_70x90mm_31x26-prt794.ipt
- C:\Users\Vincent Larson\Downloads\Universal_board_70x90mm_31x26\Universal_board_70x90mm_31x26-prt795.ipt
- C:\Users\Vincent Larson\Downloads\Universal_board_70x90mm_31x26\Universal_board_70x90mm_31x26-prt796.ipt
- C:\Users\Vincent Larson\Downloads\Universal_board_70x90mm_31x26\Universal_board_70x90mm_31x26-prt797.ipt
- C:\Users\Vincent Larson\Downloads\Universal_board_70x90mm_31x26\Universal_board_70x90mm_31x26-prt798.ipt
- C:\Users\Vincent Larson\Downloads\Universal_board_70x90mm_31x26\Universal_board_70x90mm_31x26-prt799.ipt
- C:\Users\Vincent Larson\Downloads\Universal_board_70x90mm_31x26\Universal_board_70x90mm_31x26-prt800.ipt
- C:\Users\Vincent Larson\Downloads\Universal_board_70x90mm_31x26\Universal_board_70x90mm_31x26-prt801.ipt
- C:\Users\Vincent Larson\Downloads\Universal_board_70x90mm_31x26\Universal_board_70x90mm_31x26-prt802.ipt
- C:\Users\Vincent Larson\Downloads\Universal_board_70x90mm_31x26\Universal_board_70x90mm_31x26-prt803.ipt
- C:\Users\Vincent Larson\Downloads\Universal_board_70x90mm_31x26\Universal_board_70x90mm_31x26-prt804.ipt
- C:\Users\Vincent Larson\Downloads\Universal_board_70x90mm_31x26\Universal_board_70x90mm_31x26-prt805.ipt
- C:\Users\Vincent Larson\Downloads\Universal_board_70x90mm_31x26\Universal_board_70x90mm_31x26-prt806.ipt
- C:\Users\Vincent Larson\Downloads\Universal_board_70x90mm_31x26\Universal_board_70x90mm_31x26-prt807.ipt
- C:\Users\Vincent Larson\Downloads\Universal_board_70x90mm_31x26\Universal_board_70x90mm_31x26-prt808.ipt
- C:\Users\Vincent Larson\Downloads\Universal_board_70x90mm_31x26\Universal_board_70x90mm_31x26-prt809.ipt
- C:\Users\Vincent Larson\Downloads\Universal_board_70x90mm_31x26\Universal_board_70x90mm_31x26-prt810.ipt
- C:\Users\Vincent Larson\Downloads\Universal_board_70x90mm_31x26\Universal_board_70x90mm_31x26-prt811.ipt
- C:\Users\Vincent Larson\Downloads\Universal_board_70x90mm_31x26\Universal_board_70x90mm_31x26-prt812.ipt
- C:\Users\Vincent Larson\Downloads\Universal_board_70x90mm_31x26\Universal_board_70x90mm_31x26-prt813.ipt
- C:\Users\Vincent Larson\Downloads\Universal_board_70x90mm_31x26\Universal_board_70x90mm_31x26-prt814.ipt
- C:\Users\Vincent Larson\Downloads\Universal_board_70x90mm_31x26\Universal_board_70x90mm_31x26-prt815.ipt
- C:\Users\Vincent Larson\Downloads\Universal_board_70x90mm_31x26\Universal_board_70x90mm_31x26-prt816.ipt
- C:\Users\Vincent Larson\Downloads\Universal_board_70x90mm_31x26\Universal_board_70x90mm_31x26-prt817.ipt
- C:\Users\Vincent Larson\Downloads\Universal_board_70x90mm_31x26\Universal_board_70x90mm_31x26-prt818.ipt
- C:\Users\Vincent Larson\Downloads\Universal_board_70x90mm_31x26\Universal_board_70x90mm_31x26-prt819.ipt
- C:\Users\Vincent Larson\Downloads\Universal_board_70x90mm_31x26\Universal_board_70x90mm_31x26-prt820.ipt
- C:\Users\Vincent Larson\Downloads\Universal_board_70x90mm_31x26\Universal_board_70x90mm_31x26-prt821.ipt
- C:\Users\Vincent Larson\Downloads\Universal_board_70x90mm_31x26\Universal_board_70x90mm_31x26-prt822.ipt
- C:\Users\Vincent Larson\Downloads\Universal_board_70x90mm_31x26\Universal_board_70x90mm_31x26-prt823.ipt
- C:\Users\Vincent Larson\Downloads\Universal_board_70x90mm_31x26\Universal_board_70x90mm_31x26-prt824.ipt
- C:\Users\Vincent Larson\Downloads\Universal_board_70x90mm_31x26\Universal_board_70x90mm_31x26-prt825.ipt
- C:\Users\Vincent Larson\Downloads\Universal_board_70x90mm_31x26\Universal_board_70x90mm_31x26-prt826.ipt
- C:\Users\Vincent Larson\Downloads\Universal_board_70x90mm_31x26\Universal_board_70x90mm_31x26-prt827.ipt
- C:\Users\Vincent Larson\Downloads\Universal_board_70x90mm_31x26\Universal_board_70x90mm_31x26-prt828.ipt
- C:\Users\Vincent Larson\Downloads\Universal_board_70x90mm_31x26\Universal_board_70x90mm_31x26-prt829.ipt
- C:\Users\Vincent Larson\Downloads\Universal_board_70x90mm_31x26\Universal_board_70x90mm_31x26-prt830.ipt
- C:\Users\Vincent Larson\Downloads\Universal_board_70x90mm_31x26\Universal_board_70x90mm_31x26-prt831.ipt
- C:\Users\Vincent Larson\Downloads\Universal_board_70x90mm_31x26\Universal_board_70x90mm_31x26-prt832.ipt
- C:\Users\Vincent Larson\Downloads\Universal_board_70x90mm_31x26\Universal_board_70x90mm_31x26-prt833.ipt
- C:\Users\Vincent Larson\Downloads\Universal_board_70x90mm_31x26\Universal_board_70x90mm_31x26-prt834.ipt
- C:\Users\Vincent Larson\Downloads\Universal_board_70x90mm_31x26\Universal_board_70x90mm_31x26-prt835.ipt
- C:\Users\Vincent Larson\Downloads\Universal_board_70x90mm_31x26\Universal_board_70x90mm_31x26-prt836.ipt
- C:\Users\Vincent Larson\Downloads\Universal_board_70x90mm_31x26\Universal_board_70x90mm_31x26-prt837.ipt
- C:\Users\Vincent Larson\Downloads\Universal_board_70x90mm_31x26\Universal_board_70x90mm_31x26-prt838.ipt
- C:\Users\Vincent Larson\Downloads\Universal_board_70x90mm_31x26\Universal_board_70x90mm_31x26-prt839.ipt
- C:\Users\Vincent Larson\Downloads\Universal_board_70x90mm_31x26\Universal_board_70x90mm_31x26-prt840.ipt
- C:\Users\Vincent Larson\Downloads\Universal_board_70x90mm_31x26\Universal_board_70x90mm_31x26-prt841.ipt
- C:\Users\Vincent Larson\Downloads\Universal_board_70x90mm_31x26\Universal_board_70x90mm_31x26-prt842.ipt
- C:\Users\Vincent Larson\Downloads\Universal_board_70x90mm_31x26\Universal_board_70x90mm_31x26-prt843.ipt
- C:\Users\Vincent Larson\Downloads\Universal_board_70x90mm_31x26\Universal_board_70x90mm_31x26-prt844.ipt
- C:\Users\Vincent Larson\Downloads\Universal_board_70x90mm_31x26\Universal_board_70x90mm_31x26-prt845.ipt
- C:\Users\Vincent Larson\Downloads\Universal_board_70x90mm_31x26\Universal_board_70x90mm_31x26-prt846.ipt
- C:\Users\Vincent Larson\Downloads\Universal_board_70x90mm_31x26\Universal_board_70x90mm_31x26-prt847.ipt
- C:\Users\Vincent Larson\Downloads\Universal_board_70x90mm_31x26\Universal_board_70x90mm_31x26-prt848.ipt
- C:\Users\Vincent Larson\Downloads\Universal_board_70x90mm_31x26\Universal_board_70x90mm_31x26-prt849.ipt
- C:\Users\Vincent Larson\Downloads\Universal_board_70x90mm_31x26\Universal_board_70x90mm_31x26-prt850.ipt
- C:\Users\Vincent Larson\Downloads\Universal_board_70x90mm_31x26\Universal_board_70x90mm_31x26-prt851.ipt
- C:\Users\Vincent Larson\Downloads\Universal_board_70x90mm_31x26\Universal_board_70x90mm_31x26-prt852.ipt
- C:\Users\Vincent Larson\Downloads\Universal_board_70x90mm_31x26\Universal_board_70x90mm_31x26-prt853.ipt
- C:\Users\Vincent Larson\Downloads\Universal_board_70x90mm_31x26\Universal_board_70x90mm_31x26-prt854.ipt
- C:\Users\Vincent Larson\Downloads\Universal_board_70x90mm_31x26\Universal_board_70x90mm_31x26-prt855.ipt
- C:\Users\Vincent Larson\Downloads\Universal_board_70x90mm_31x26\Universal_board_70x90mm_31x26-prt856.ipt
- C:\Users\Vincent Larson\Downloads\Universal_board_70x90mm_31x26\Universal_board_70x90mm_31x26-prt857.ipt
- C:\Users\Vincent Larson\Downloads\Universal_board_70x90mm_31x26\Universal_board_70x90mm_31x26-prt858.ipt
- C:\Users\Vincent Larson\Downloads\Universal_board_70x90mm_31x26\Universal_board_70x90mm_31x26-prt859.ipt
- C:\Users\Vincent Larson\Downloads\Universal_board_70x90mm_31x26\Universal_board_70x90mm_31x26-prt860.ipt
- C:\Users\Vincent Larson\Downloads\Universal_board_70x90mm_31x26\Universal_board_70x90mm_31x26-prt861.ipt
- C:\Users\Vincent Larson\Downloads\Universal_board_70x90mm_31x26\Universal_board_70x90mm_31x26-prt862.ipt
- C:\Users\Vincent Larson\Downloads\Universal_board_70x90mm_31x26\Universal_board_70x90mm_31x26-prt863.ipt
- C:\Users\Vincent Larson\Downloads\Universal_board_70x90mm_31x26\Universal_board_70x90mm_31x26-prt864.ipt
- C:\Users\Vincent Larson\Downloads\Universal_board_70x90mm_31x26\Universal_board_70x90mm_31x26-prt865.ipt
- C:\Users\Vincent Larson\Downloads\Universal_board_70x90mm_31x26\Universal_board_70x90mm_31x26-prt866.ipt
- C:\Users\Vincent Larson\Downloads\Universal_board_70x90mm_31x26\Universal_board_70x90mm_31x26-prt867.ipt
- C:\Users\Vincent Larson\Downloads\Universal_board_70x90mm_31x26\Universal_board_70x90mm_31x26-prt868.ipt
- C:\Users\Vincent Larson\Downloads\Universal_board_70x90mm_31x26\Universal_board_70x90mm_31x26-prt869.ipt
- C:\Users\Vincent Larson\Downloads\Universal_board_70x90mm_31x26\Universal_board_70x90mm_31x26-prt870.ipt
- C:\Users\Vincent Larson\Downloads\Universal_board_70x90mm_31x26\Universal_board_70x90mm_31x26-prt871.ipt
- C:\Users\Vincent Larson\Downloads\Universal_board_70x90mm_31x26\Universal_board_70x90mm_31x26-prt872.ipt
- C:\Users\Vincent Larson\Downloads\Universal_board_70x90mm_31x26\Universal_board_70x90mm_31x26-prt873.ipt
- C:\Users\Vincent Larson\Downloads\Universal_board_70x90mm_31x26\Universal_board_70x90mm_31x26-prt874.ipt
- C:\Users\Vincent Larson\Downloads\Universal_board_70x90mm_31x26\Universal_board_70x90mm_31x26-prt875.ipt
- C:\Users\Vincent Larson\Downloads\Universal_board_70x90mm_31x26\Universal_board_70x90mm_31x26-prt876.ipt
- C:\Users\Vincent Larson\Downloads\Universal_board_70x90mm_31x26\Universal_board_70x90mm_31x26-prt877.ipt
- C:\Users\Vincent Larson\Downloads\Universal_board_70x90mm_31x26\Universal_board_70x90mm_31x26-prt878.ipt
- C:\Users\Vincent Larson\Downloads\Universal_board_70x90mm_31x26\Universal_board_70x90mm_31x26-prt879.ipt
- C:\Users\Vincent Larson\Downloads\Universal_board_70x90mm_31x26\Universal_board_70x90mm_31x26-prt880.ipt
- C:\Users\Vincent Larson\Downloads\Universal_board_70x90mm_31x26\Universal_board_70x90mm_31x26-prt881.ipt
- C:\Users\Vincent Larson\Downloads\Universal_board_70x90mm_31x26\Universal_board_70x90mm_31x26-prt882.ipt
- C:\Users\Vincent Larson\Downloads\Universal_board_70x90mm_31x26\Universal_board_70x90mm_31x26-prt883.ipt
- C:\Users\Vincent Larson\Downloads\Universal_board_70x90mm_31x26\Universal_board_70x90mm_31x26-prt884.ipt
- C:\Users\Vincent Larson\Downloads\Universal_board_70x90mm_31x26\Universal_board_70x90mm_31x26-prt885.ipt
- C:\Users\Vincent Larson\Downloads\Universal_board_70x90mm_31x26\Universal_board_70x90mm_31x26-prt886.ipt
- C:\Users\Vincent Larson\Downloads\Universal_board_70x90mm_31x26\Universal_board_70x90mm_31x26-prt887.ipt
- C:\Users\Vincent Larson\Downloads\Universal_board_70x90mm_31x26\Universal_board_70x90mm_31x26-prt888.ipt
- C:\Users\Vincent Larson\Downloads\Universal_board_70x90mm_31x26\Universal_board_70x90mm_31x26-prt889.ipt
- C:\Users\Vincent Larson\Downloads\Universal_board_70x90mm_31x26\Universal_board_70x90mm_31x26-prt890.ipt
- C:\Users\Vincent Larson\Downloads\Universal_board_70x90mm_31x26\Universal_board_70x90mm_31x26-prt891.ipt
- C:\Users\Vincent Larson\Downloads\Universal_board_70x90mm_31x26\Universal_board_70x90mm_31x26-prt892.ipt
- C:\Users\Vincent Larson\Downloads\Universal_board_70x90mm_31x26\Universal_board_70x90mm_31x26-prt893.ipt
- C:\Users\Vincent Larson\Downloads\Universal_board_70x90mm_31x26\Universal_board_70x90mm_31x26-prt894.ipt
- C:\Users\Vincent Larson\Downloads\Universal_board_70x90mm_31x26\Universal_board_70x90mm_31x26-prt895.ipt
- C:\Users\Vincent Larson\Downloads\Universal_board_70x90mm_31x26\Universal_board_70x90mm_31x26-prt896.ipt
- C:\Users\Vincent Larson\Downloads\Universal_board_70x90mm_31x26\Universal_board_70x90mm_31x26-prt897.ipt
- C:\Users\Vincent Larson\Downloads\Universal_board_70x90mm_31x26\Universal_board_70x90mm_31x26-prt898.ipt
- C:\Users\Vincent Larson\Downloads\Universal_board_70x90mm_31x26\Universal_board_70x90mm_31x26-prt899.ipt
- C:\Users\Vincent Larson\Downloads\Universal_board_70x90mm_31x26\Universal_board_70x90mm_31x26-prt900.ipt
- C:\Users\Vincent Larson\Downloads\Universal_board_70x90mm_31x26\Universal_board_70x90mm_31x26-prt901.ipt
- C:\Users\Vincent Larson\Downloads\Universal_board_70x90mm_31x26\Universal_board_70x90mm_31x26-prt902.ipt
- C:\Users\Vincent Larson\Downloads\Universal_board_70x90mm_31x26\Universal_board_70x90mm_31x26-prt903.ipt
- C:\Users\Vincent Larson\Downloads\Universal_board_70x90mm_31x26\Universal_board_70x90mm_31x26-prt904.ipt
- C:\Users\Vincent Larson\Downloads\Universal_board_70x90mm_31x26\Universal_board_70x90mm_31x26-prt905.ipt
- C:\Users\Vincent Larson\Downloads\Universal_board_70x90mm_31x26\Universal_board_70x90mm_31x26-prt906.ipt
## Components (907 placed, 907 different names)
1. Universal_board_70x90mm_31x26-prt0
2. Universal_board_70x90mm_31x26-prt1
3. Universal_board_70x90mm_31x26-prt2
4. Universal_board_70x90mm_31x26-prt3
5. Universal_board_70x90mm_31x26-prt4
6. Universal_board_70x90mm_31x26-prt5
7. Universal_board_70x90mm_31x26-prt6
8. Universal_board_70x90mm_31x26-prt7
9. Universal_board_70x90mm_31x26-prt8
10. Universal_board_70x90mm_31x26-prt9
11. Universal_board_70x90mm_31x26-prt10
12. Universal_board_70x90mm_31x26-prt11
13. Universal_board_70x90mm_31x26-prt12
14. Universal_board_70x90mm_31x26-prt13
15. Universal_board_70x90mm_31x26-prt14
16. Universal_board_70x90mm_31x26-prt15
17. Universal_board_70x90mm_31x26-prt16
18. Universal_board_70x90mm_31x26-prt17
19. Universal_board_70x90mm_31x26-prt18
20. Universal_board_70x90mm_31x26-prt19
21. Universal_board_70x90mm_31x26-prt20
22. Universal_board_70x90mm_31x26-prt21
23. Universal_board_70x90mm_31x26-prt22
24. Universal_board_70x90mm_31x26-prt23
25. Universal_board_70x90mm_31x26-prt24
26. Universal_board_70x90mm_31x26-prt25
27. Universal_board_70x90mm_31x26-prt26
28. Universal_board_70x90mm_31x26-prt27
29. Universal_board_70x90mm_31x26-prt28
30. Universal_board_70x90mm_31x26-prt29
31. Universal_board_70x90mm_31x26-prt30
32. Universal_board_70x90mm_31x26-prt31
33. Universal_board_70x90mm_31x26-prt32
34. Universal_board_70x90mm_31x26-prt33
35. Universal_board_70x90mm_31x26-prt34
36. Universal_board_70x90mm_31x26-prt35
37. Universal_board_70x90mm_31x26-prt36
38. Universal_board_70x90mm_31x26-prt37
39. Universal_board_70x90mm_31x26-prt38
40. Universal_board_70x90mm_31x26-prt39
41. Universal_board_70x90mm_31x26-prt40
42. Universal_board_70x90mm_31x26-prt41
43. Universal_board_70x90mm_31x26-prt42
44. Universal_board_70x90mm_31x26-prt43
45. Universal_board_70x90mm_31x26-prt44
46. Universal_board_70x90mm_31x26-prt45
47. Universal_board_70x90mm_31x26-prt46
48. Universal_board_70x90mm_31x26-prt47
49. Universal_board_70x90mm_31x26-prt48
50. Universal_board_70x90mm_31x26-prt49
51. Universal_board_70x90mm_31x26-prt50
52. Universal_board_70x90mm_31x26-prt51
53. Universal_board_70x90mm_31x26-prt52